# Autodesk Inventor assembly: Grabber
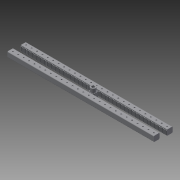
[picture p0: Inventor's stored thumbnail of the model, 180x180]
Saved by Autodesk Inventor 2015 (Build 190159000, 159)
## iProperties
Created: 2015-01-14
Part Number: Grabber
Document SubType Name: Assembly
Designer: Jarod
Author: Jarod
## Documents named in this file (4)
- D:\Robotics\FRC\2015\CAD\Robot\Grabber\Grabber.iam
- D:\Robotics\FRC\2015\CAD\Robot\Grabber\c-channel.ipt
- D:\Robotics\FRC\2015\CAD\Robot\Grabber\rack.ipt
- D:\Robotics\FRC\2015\CAD\Robot\Grabber\pinion.ipt
## Components (5 placed, 3 different names)
1. c-channel:1 — Mate:1, Flush:4, Mate:2, Flush:6, Mate:5, Mate:7, Flush:7, Mate:8, Mate:9, Flush:8
2. c-channel:2 — Mate:3, Flush:5, Mate:4, Mate:6, Mate:7, Flush:7
3. rack:1 — Mate:1, Flush:4, Mate:2
4. rack:2 — Mate:3, Flush:5, Mate:4
5. pinion:1 — Flush:6, Mate:5, Mate:6
## Relationships (14: Mate 9, Flush 5)
- Mate:1: c-channel:1 ↔ rack:1
- Flush:4: c-channel:1 ↔ rack:1
- Mate:2: c-channel:1 ↔ rack:1
- Mate:3: c-channel:2 ↔ rack:2
- Flush:5: c-channel:2 ↔ rack:2
- Mate:4: c-channel:2 ↔ rack:2
- Flush:6 (0.7937 mm): c-channel:1 ↔ pinion:1
- Mate:5 (15.875 mm): c-channel:1 ↔ pinion:1
- Mate:6 (15.875 mm): c-channel:2 ↔ pinion:1
- Mate:7 (31.75 mm): c-channel:1 ↔ c-channel:2
- Flush:7: c-channel:1 ↔ c-channel:2
- Mate:8: c-channel:1
- Mate:9: c-channel:1
- Flush:8: c-channel:1
